# Autodesk Inventor assembly: 00 INSTALLATION
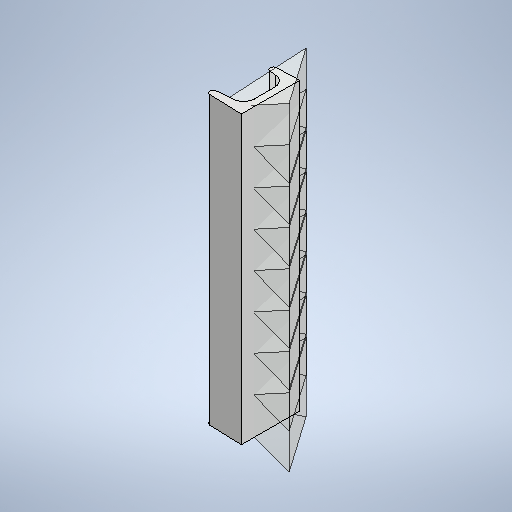
[picture p0: Inventor's stored thumbnail of the model, 512x512]
Saved by Autodesk Inventor 2025 (Build 290162000, 162)
## iProperties
Created: 2026-03-19
Part Number: 00 INSTALLATION
Document SubType Name: Assembly
Designer: steve
Author: steve
## Documents named in this file (3)
- C:\Users\steve\Documents\Business\BunkScanner\Design\3D\00 INSTALLATION.iam
- C:\Users\steve\Documents\Business\BunkScanner\Design\3D\Bunk 1.ipt
- C:\Users\steve\Documents\Business\BunkScanner\Design\3D\vl53l7cx-carrier-model.iam
## Components (9 placed, 2 different names)
1. Bunk 1:1 — Flush:1, Flush:2, Flush:3, Mate:1, Mate:2
2. vl53l7cx-carrier-model:1 — Mate:1, Angle:1, Mate:2
3. vl53l7cx-carrier-model:2
4. vl53l7cx-carrier-model:3
5. vl53l7cx-carrier-model:4
6. vl53l7cx-carrier-model:5
7. vl53l7cx-carrier-model:6
8. vl53l7cx-carrier-model:7
9. vl53l7cx-carrier-model:8
## Component patterns: (8 elements, first: vl53l7cx-carrier-model:1)
## Relationships (6: Flush 3, Mate 2, Angle 1)
- Flush:1: Bunk 1:1
- Flush:2: Bunk 1:1
- Flush:3: Bunk 1:1
- Mate:1 (100 mm): Bunk 1:1 ↔ vl53l7cx-carrier-model:1
- Angle:1 (55 deg): vl53l7cx-carrier-model:1
- Mate:2 (-300 mm): Bunk 1:1 ↔ vl53l7cx-carrier-model:1
